# Autodesk Inventor assembly: Tool_DC_007
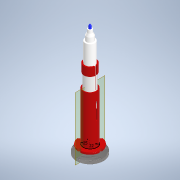
[picture p0: Inventor's stored thumbnail of the model, 180x180]
Saved by Autodesk Inventor 2022 (Build 260153000, 153)
## iProperties
Created: 2022-09-01
Part Number: Tool_DC_007
Document SubType Name: Assembly
Designer: Asus
Author: Asus
## Documents named in this file (4)
- C:\Users\Asus\Desktop\Robotica\CAD-Robotica\Tool_DC_007.iam
- C:\Users\Asus\Desktop\Robotica\CAD-Robotica\Base.ipt
- C:\Users\Asus\Desktop\Robotica\CAD-Robotica\Cilindro.ipt
- C:\Users\Asus\Desktop\Robotica\CAD-Robotica\MArcador.ipt
## Components (3 placed, 3 different names)
1. Base:1 — Mate:1, Mate:2, Mate:3, Flush:5, Mate:5, Mate:6, Mate:8, Mate:9, Flush:6
2. Cilindro:2 — Flush:5, Mate:5, Mate:7, Mate:9
3. MArcador:1 — Mate:6, Mate:7, Mate:8
## Relationships (10: Mate 8, Flush 2)
- Mate:1: Base:1
- Mate:2: Base:1
- Mate:3: Base:1
- Flush:5: Base:1 ↔ Cilindro:2
- Mate:5: Base:1 ↔ Cilindro:2
- Mate:6: Base:1 ↔ MArcador:1
- Mate:7: Cilindro:2 ↔ MArcador:1
- Mate:8: Base:1 ↔ MArcador:1
- Mate:9 (40 mm): Base:1 ↔ Cilindro:2
- Flush:6: Base:1
